# Autodesk Inventor assembly: ServoControllerAssembly
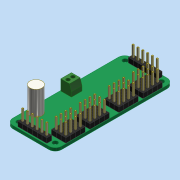
[picture p0: Inventor's stored thumbnail of the model, 180x180]
Saved by Autodesk Inventor 2017 (Build 210142000, 142)
## iProperties
Created: 2017-01-25
Part Number: ServoControllerAssembly
Document SubType Name: Assembly
Designer: techn
Mass: 22.6796 g
Surface Area: 84.6883 cm^2
Volume: 4.03545 cm^3
Author: techn
## Documents named in this file (6)
- G:\Projects\Submarine\Submarine-project\CAD\midships\ElectronicsSection\ServoController\ServoControllerAssembly.iam
- G:\Projects\Submarine\Submarine-project\CAD\midships\ElectronicsSection\ServoController\3PinBlock.iam
- G:\Projects\Submarine\Submarine-project\CAD\midships\ElectronicsSection\ServoController\6PinBlock.iam
- G:\Projects\Submarine\Submarine-project\CAD\midships\ElectronicsSection\ServoController\MainPCB.ipt
- G:\Projects\Submarine\Submarine-project\CAD\midships\ElectronicsSection\ServoController\Capacitor.ipt
- G:\Projects\Submarine\Submarine-project\CAD\midships\ElectronicsSection\ServoController\connector.ipt
## Components (21 placed, 5 different names)
1. 6PinBlock:1 [sub-assembly] — Mate:2, Flush:3, Flush:4
2. MainPCB:1 — Flush:1, Flush:2, Mate:1, Mate:2, Flush:4, Mate:3, Flush:5, Flush:6, Mate:4, Tangent:1, Tangent:2, Mate:5, Flush:7, Flush:8
3. 6PinBlock:2 [sub-assembly] — Flush:1, Flush:2, Mate:1, Flush:3
4. Capacitor:1 — Mate:4, Tangent:1, Tangent:2
5. connector:1 — Mate:5, Flush:7, Flush:8
6. 3PinBlock:1 [sub-assembly] — Mate:3, Flush:5, Flush:6
7. 3PinBlock:2 [sub-assembly]
8. 3PinBlock:3 [sub-assembly]
9. 3PinBlock:4 [sub-assembly]
10. 3PinBlock:5 [sub-assembly]
11. 3PinBlock:6 [sub-assembly]
12. 3PinBlock:7 [sub-assembly]
13. 3PinBlock:8 [sub-assembly]
14. 3PinBlock:9 [sub-assembly]
15. 3PinBlock:10 [sub-assembly]
16. 3PinBlock:11 [sub-assembly]
17. 3PinBlock:12 [sub-assembly]
18. 3PinBlock:13 [sub-assembly]
19. 3PinBlock:14 [sub-assembly]
20. 3PinBlock:15 [sub-assembly]
21. 3PinBlock:16 [sub-assembly]
## Component patterns: (2 elements), (2 elements), Component Pattern 2:2 (2 elements), (4 elements, first: 3PinBlock:1), Component Pattern 1:2 (4 elements), Component Pattern 1:3 (4 elements), Component Pattern 1:4 (4 elements)
## Relationships (15: Flush 8, Mate 5, Tangent 2)
- Flush:1 (0.762 mm): MainPCB:1 ↔ 6PinBlock:2
- Flush:2 (5.207 mm): MainPCB:1 ↔ 6PinBlock:2
- Mate:1: MainPCB:1 ↔ 6PinBlock:2
- Mate:2: 6PinBlock:1 ↔ MainPCB:1
- Flush:3: 6PinBlock:1 ↔ 6PinBlock:2
- Flush:4 (0.762 mm): 6PinBlock:1 ↔ MainPCB:1
- Mate:3: MainPCB:1 ↔ 3PinBlock:1
- Flush:5 (0.254 mm): MainPCB:1 ↔ 3PinBlock:1
- Flush:6 (5.842 mm): MainPCB:1 ↔ 3PinBlock:1
- Mate:4: MainPCB:1 ↔ Capacitor:1
- Tangent:1 (0.254 mm): MainPCB:1 ↔ Capacitor:1
- Tangent:2 (8.89 mm): MainPCB:1 ↔ Capacitor:1
- Mate:5: MainPCB:1 ↔ connector:1
- Flush:7 (0.254 mm): MainPCB:1 ↔ connector:1
- Flush:8 (28.321 mm): MainPCB:1 ↔ connector:1
